# Autodesk Inventor assembly: 1-112
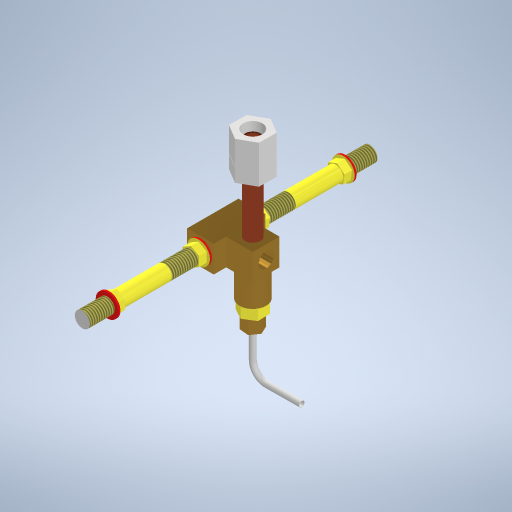
[picture p0: Inventor's stored thumbnail of the model, 512x512]
Saved by Autodesk Inventor 2024.2 (Build 282272000, 272)
## iProperties
Created: 2024-11-02
Part Number: 1-112
Document SubType Name: Assembly
Designer: melim
Author: melim
## Documents named in this file (8)
- C:\Users\melim\OneDrive\Desktop\ENSAMBLES\1-112\1-112.iam
- C:\Users\melim\OneDrive\Desktop\ENSAMBLES\1-112\HUDSON-1-45.ipt
- C:\Users\melim\OneDrive\Desktop\ENSAMBLES\1-112\HUDSON-1-47.ipt
- C:\Users\melim\OneDrive\Desktop\ENSAMBLES\1-112\HUDSON-1-108.ipt
- C:\Users\melim\OneDrive\Desktop\ENSAMBLES\1-112\HUDSON-1-49\HUDSON-1-49.ipt
- C:\Users\melim\OneDrive\Desktop\ENSAMBLES\1-112\HUDSON1-46.ipt
- C:\Users\melim\OneDrive\Desktop\ENSAMBLES\1-112\Hudson 1-69.iam
- C:\Users\melim\OneDrive\Desktop\ENSAMBLES\1-112\Hudson 1-70.ipt
## Components (8 placed, 7 different names)
1. HUDSON-1-45:1 — Mate:1, Mate:3, Mate:6, Mate:7, Mate:8, Mate:9, Mate:10, Mate:11
2. HUDSON-1-47:1 — Mate:1, Mate:2, Mate:3, Mate:4, Mate:5
3. HUDSON-1-108:1 — Mate:2, Mate:4, Mate:5
4. HUDSON-1-49:1 — Mate:6, Mate:7
5. HUDSON-1-49:2 — Mate:8, Mate:9
6. HUDSON1-46:1 — Mate:10, Mate:11, Mate:12, Mate:13, Mate:15
7. Hudson 1-69:1 [sub-assembly] — Mate:12, Mate:13, Mate:14
8. Hudson 1-70:1 — Mate:14, Mate:15
## Relationships (15: Mate 15)
- Mate:1: HUDSON-1-45:1 ↔ HUDSON-1-47:1
- Mate:2: HUDSON-1-47:1 ↔ HUDSON-1-108:1
- Mate:3: HUDSON-1-45:1 ↔ HUDSON-1-47:1
- Mate:4: HUDSON-1-47:1 ↔ HUDSON-1-108:1
- Mate:5: HUDSON-1-47:1 ↔ HUDSON-1-108:1
- Mate:6: HUDSON-1-45:1 ↔ HUDSON-1-49:1
- Mate:7: HUDSON-1-45:1 ↔ HUDSON-1-49:1
- Mate:8: HUDSON-1-45:1 ↔ HUDSON-1-49:2
- Mate:9: HUDSON-1-45:1 ↔ HUDSON-1-49:2
- Mate:10: HUDSON-1-45:1 ↔ HUDSON1-46:1
- Mate:11: HUDSON-1-45:1 ↔ HUDSON1-46:1
- Mate:12: HUDSON1-46:1 ↔ Hudson 1-69:1
- Mate:13: HUDSON1-46:1 ↔ Hudson 1-69:1
- Mate:14: Hudson 1-69:1 ↔ Hudson 1-70:1
- Mate:15: HUDSON1-46:1 ↔ Hudson 1-70:1
